# Autodesk Inventor assembly: upper_fin1
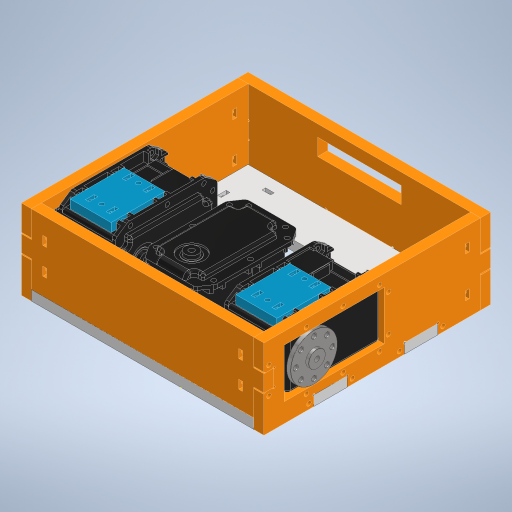
[picture p0: Inventor's stored thumbnail of the model, 512x512]
Saved by Autodesk Inventor 2024 (Build 280153000, 153)
## iProperties
Created: 2024-09-14
Part Number: upper_fin1
Document SubType Name: Assembly
Designer: jmha0
Author: jmha0
## Documents named in this file (8)
- C:\Users\jmha0\OneDrive\바탕 화면\19th_intern_hjm_fight_robot\Upper_Body\Upper\upper_fin1.iam
- C:\Users\jmha0\OneDrive\바탕 화면\19th_intern_hjm_fight_robot\Upper_Body\Upper\frame_upper1.ipt
- C:\Users\jmha0\OneDrive\바탕 화면\19th_intern_hjm_fight_robot\hardware\ROBOTIS(Inventor 2024 ver.)\다이나믹셀\MX-64T.ipt
- C:\Users\jmha0\OneDrive\바탕 화면\19th_intern_hjm_fight_robot\hardware\ROBOTIS(Inventor 2024 ver.)\혼\64-106Horn.ipt
- C:\Users\jmha0\OneDrive\바탕 화면\19th_intern_hjm_fight_robot\Upper_Body\Upper\frame_upper2.ipt
- C:\Users\jmha0\OneDrive\바탕 화면\19th_intern_hjm_fight_robot\Upper_Body\Upper\frame_upper3.ipt
- C:\Users\jmha0\OneDrive\바탕 화면\19th_intern_hjm_fight_robot\Upper_Body\Upper\frame_upper4.ipt
- C:\Users\jmha0\OneDrive\바탕 화면\19th_intern_hjm_fight_robot\Upper_Body\Upper\3D_upper_to_head1.ipt
## Components (13 placed, 7 different names)
1. frame_upper1:1 — 삽입:4, 삽입:5, 삽입:6, 삽입:7, 삽입:8, 삽입:9, 삽입:10, 삽입:23, 삽입:24
2. MX-64T:1 — 삽입:1, 삽입:4, 삽입:5, 삽입:6
3. MX-64T:2 — 삽입:2, 삽입:16, 삽입:17, 삽입:18, 삽입:19, 삽입:27, 삽입:28
4. MX-64T:3 — 삽입:12, 삽입:13, 삽입:14, 삽입:15, 삽입:25, 삽입:26
5. 64-106Horn:1 — 삽입:1
6. 64-106Horn:2 — 삽입:12
7. 64-106Horn:3 — 삽입:2
8. frame_upper2:1 — 삽입:7, 삽입:8, 삽입:13, 삽입:14, 삽입:15, 삽입:20, 삽입:21
9. frame_upper2:2 — 삽입:9, 삽입:10, 삽입:16, 삽입:17, 삽입:18, 삽입:19, 삽입:22
10. frame_upper3:1 — 삽입:20, 삽입:21, 삽입:22
11. frame_upper4:1 — 삽입:23, 삽입:24
12. 3D_upper_to_head1:1 — 삽입:27, 삽입:28
13. 3D_upper_to_head1:2 — 삽입:25, 삽입:26
## Relationships (26: Insert 26)
- 삽입:1 [Insert] (0.1 mm): MX-64T:1 ↔ 64-106Horn:1
- 삽입:2 [Insert] (0.1 mm): MX-64T:2 ↔ 64-106Horn:3
- 삽입:4 [Insert]: frame_upper1:1 ↔ MX-64T:1
- 삽입:5 [Insert]: frame_upper1:1 ↔ MX-64T:1
- 삽입:6 [Insert]: frame_upper1:1 ↔ MX-64T:1
- 삽입:7 [Insert]: frame_upper1:1 ↔ frame_upper2:1
- 삽입:8 [Insert]: frame_upper1:1 ↔ frame_upper2:1
- 삽입:9 [Insert]: frame_upper1:1 ↔ frame_upper2:2
- 삽입:10 [Insert]: frame_upper1:1 ↔ frame_upper2:2
- 삽입:12 [Insert] (0.1 mm): MX-64T:3 ↔ 64-106Horn:2
- 삽입:13 [Insert]: MX-64T:3 ↔ frame_upper2:1
- 삽입:14 [Insert]: MX-64T:3 ↔ frame_upper2:1
- 삽입:15 [Insert]: MX-64T:3 ↔ frame_upper2:1
- 삽입:16 [Insert]: MX-64T:2 ↔ frame_upper2:2
- 삽입:17 [Insert]: MX-64T:2 ↔ frame_upper2:2
- 삽입:18 [Insert]: MX-64T:2 ↔ frame_upper2:2
- 삽입:19 [Insert]: MX-64T:2 ↔ frame_upper2:2
- 삽입:20 [Insert]: frame_upper2:1 ↔ frame_upper3:1
- 삽입:21 [Insert]: frame_upper2:1 ↔ frame_upper3:1
- 삽입:22 [Insert]: frame_upper2:2 ↔ frame_upper3:1
- 삽입:23 [Insert]: frame_upper1:1 ↔ frame_upper4:1
- 삽입:24 [Insert]: frame_upper1:1 ↔ frame_upper4:1
- 삽입:25 [Insert] (2 mm): MX-64T:3 ↔ 3D_upper_to_head1:2
- 삽입:26 [Insert] (2 mm): MX-64T:3 ↔ 3D_upper_to_head1:2
- 삽입:27 [Insert] (2 mm): MX-64T:2 ↔ 3D_upper_to_head1:1
- 삽입:28 [Insert] (2 mm): MX-64T:2 ↔ 3D_upper_to_head1:1
